# Autodesk Inventor assembly: Camera
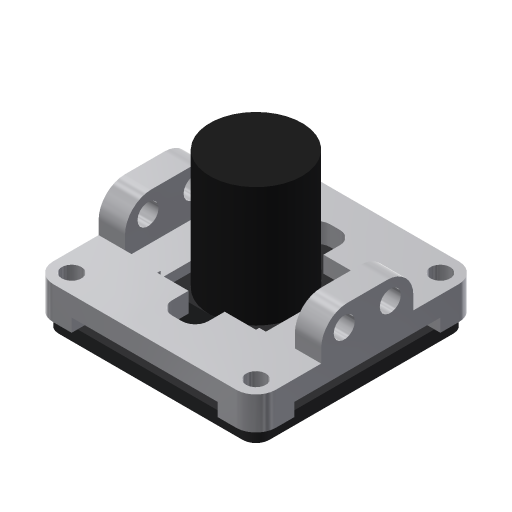
[picture p0: Inventor's stored thumbnail of the model, 512x512]
Saved by Autodesk Inventor 2023.2 (Build 272271000, 271)
## iProperties
Created: 2021-07-30
Part Number: Camera
Material: 일반
Document SubType Name: Assembly
Designer: user
Mass: 14.455 g
Surface Area: 73.477 cm^2
Volume: 9.10847 cm^3
Density: 1.58698 g/cm^3
Author: user
## Documents named in this file (3)
- \\192.168.0.49\robit_ftp3\999 Private Folder\15기 이은수\2021 manipulator (국방로봇)\Gripper (국방로봇)\Camera.iam
- \\192.168.0.49\robit_ftp3\999 Private Folder\15기 이은수\2021 manipulator (국방로봇)\Gripper (국방로봇)\Camera.ipt
- \\192.168.0.49\robit_ftp3\999 Private Folder\15기 이은수\2021 manipulator (국방로봇)\Gripper (국방로봇)\Camera_Cover.ipt
## Components (2 placed, 2 different names)
1. Camera:1 — 삽입:1, 삽입:2, 삽입:5, 삽입:6
2. Camera_Cover:1 — 삽입:1, 삽입:2, 삽입:5, 삽입:6
## Relationships (4: Insert 4)
- 삽입:1 [Insert]: Camera:1 ↔ Camera_Cover:1
- 삽입:2 [Insert]: Camera:1 ↔ Camera_Cover:1
- 삽입:5 [Insert]: Camera:1 ↔ Camera_Cover:1
- 삽입:6 [Insert]: Camera:1 ↔ Camera_Cover:1
